# Autodesk Inventor assembly: ASY дренаж угольные
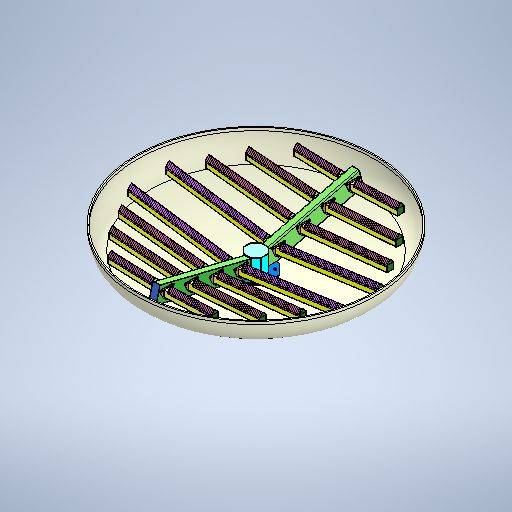
[picture p0: Inventor's stored thumbnail of the model, 512x512]
Saved by Autodesk Inventor 2025.1 (Build 291241020, 241B)
## iProperties
Created: 2024-12-09
Part Number: ASY дренаж угольные
Document SubType Name: Assembly
Designer: user
Author: user
## Documents named in this file (15)
- C:\Users\user\YandexDisk-badmisterfox\home pc\Inventor\filter-distribution-system\ASY BOTTOM filter distribution system.iam
- C:\Users\user\YandexDisk-badmisterfox\home pc\Inventor\filter-distribution-system\drain flange.ipt
- C:\Users\user\YandexDisk-badmisterfox\home pc\Inventor\filter-distribution-system\dished head.ipt
- C:\Users\user\YandexDisk-badmisterfox\home pc\Inventor\filter-distribution-system\DS-B-102 ridge bottom.ipt
- C:\Users\user\YandexDisk-badmisterfox\home pc\Inventor\filter-distribution-system\DS-B-101 Axis.ipt
- C:\Users\user\YandexDisk-badmisterfox\home pc\Inventor\filter-distribution-system\DS-B-104 ridge end cap.ipt
- C:\Users\user\YandexDisk-badmisterfox\home pc\Inventor\filter-distribution-system\DS-B-103 Ridge top.ipt
- C:\Users\user\YandexDisk-badmisterfox\home pc\Inventor\filter-distribution-system\ASY DS-B beam 1.iam
- C:\Users\user\YandexDisk-badmisterfox\home pc\Inventor\filter-distribution-system\000 DS-B dimentions.ipt
- C:\Users\user\YandexDisk-badmisterfox\home pc\Inventor\filter-distribution-system\111 DS-B outer tube.ipt
- C:\Users\user\YandexDisk-badmisterfox\home pc\Inventor\filter-distribution-system\110 DS-B drain sustem flange.ipt
- C:\Users\user\YandexDisk-badmisterfox\home pc\Inventor\filter-distribution-system\ASY DS-B beam 2.iam
- C:\Users\user\YandexDisk-badmisterfox\home pc\Inventor\filter-distribution-system\ASY DS-B beam 3.iam
- C:\Users\user\YandexDisk-badmisterfox\home pc\Inventor\filter-distribution-system\ASY DS-B beam 4.iam
- C:\Users\user\YandexDisk-badmisterfox\home pc\Inventor\filter-distribution-system\210 DS-B Axis cap.ipt
## Components (30 placed, 16 different names)
1. 000 DS-B dimentions.ipt:1
2. dished head.ipt:1 — Mate:4, Flush:3, Flush:4, Rigid:36
3. MNT-CDF-501 box.ipt:1 — Mate:5, Flush:5, Mate:6, Rigid:42, Rigid:43, Rigid:44, Rigid:45, Rigid:46
4. drain flange.ipt:1 — Rigid:37
5. MNT-CDF-503  main tube 1.ipt:1 — Rigid:39, Mate:7, Rigid:50
6. MNT-CDF-503  main tube 1.ipt:2 — Mate:5, Rigid:38
7. MNT-CDF-501 box.ipt:2 — Mate:7, Mate:8, Mate:9, Rigid:47, Rigid:52, Rigid:57, Rigid:58, Rigid:59
8. MNT-CDF-602 CAP.ipt:1 — Rigid:49
9. MNT-CDF-602 CAP.ipt:2 — Rigid:48
10. MNT-CDF-603 CAP.ipt:2 — Rigid:46, Rigid:49, Rigid:54, Rigid:55, Rigid:56, Rigid:63
11. ASY CDF 1100 beam 1.iam:1 [sub-assembly] — Rigid:42
12. 000 DS-B outer tube.ipt:1 — Rigid:36, Rigid:37
13. 110 DS-B drain sustem flange.ipt:1 — Mate:6, Rigid:38, Rigid:39, Mate:8
14. ASY DS-B beam 2:1 [sub-assembly] — Rigid:43
15. ASY DS-B beam 3:1 [sub-assembly] — Rigid:44
16. ASY DS-B beam 4:1 [sub-assembly] — Rigid:45
17. MNT-CDF-603 CAP:3 — Rigid:47, Rigid:48, Rigid:53, Rigid:60, Rigid:61, Rigid:62
18. 210 DS-B Axis cap:1 — Rigid:50
19. ASY DS-B beam 1:2 [sub-assembly] — Rigid:63
20. ASY DS-B beam 1:3 [sub-assembly] — Rigid:52
21. ASY DS-B beam 1:4 [sub-assembly] — Rigid:53
22. ASY DS-B beam 2:2 [sub-assembly] — Rigid:54
23. ASY DS-B beam 3:2 [sub-assembly] — Rigid:55
24. ASY DS-B beam 4:2 [sub-assembly] — Rigid:56
25. ASY DS-B beam 2:3 [sub-assembly] — Rigid:57
26. ASY DS-B beam 3:3 [sub-assembly] — Rigid:58
27. ASY DS-B beam 4:3 [sub-assembly] — Rigid:59
28. ASY DS-B beam 2:4 [sub-assembly] — Rigid:60
29. ASY DS-B beam 3:4 [sub-assembly] — Rigid:61
30. ASY DS-B beam 4:4 [sub-assembly] — Rigid:62
## Relationships (34: WeldJoint 25, Mate 6, Flush 3)
- Mate:4: dished head.ipt:1
- Flush:3: dished head.ipt:1
- Flush:4: dished head.ipt:1
- Rigid:36 [WeldJoint]: dished head.ipt:1 ↔ 000 DS-B outer tube.ipt:1
- Rigid:37 [WeldJoint]: drain flange.ipt:1 ↔ 000 DS-B outer tube.ipt:1
- Mate:5: MNT-CDF-501 box.ipt:1 ↔ MNT-CDF-503  main tube 1.ipt:2
- Flush:5: MNT-CDF-501 box.ipt:1
- Mate:6: MNT-CDF-501 box.ipt:1 ↔ 110 DS-B drain sustem flange.ipt:1
- Rigid:38 [WeldJoint]: MNT-CDF-503  main tube 1.ipt:2 ↔ 110 DS-B drain sustem flange.ipt:1
- Rigid:39 [WeldJoint]: MNT-CDF-503  main tube 1.ipt:1 ↔ 110 DS-B drain sustem flange.ipt:1
- Mate:7: MNT-CDF-503  main tube 1.ipt:1 ↔ MNT-CDF-501 box.ipt:2
- Mate:8: MNT-CDF-501 box.ipt:2 ↔ 110 DS-B drain sustem flange.ipt:1
- Mate:9: MNT-CDF-501 box.ipt:2
- Rigid:42 [WeldJoint]: MNT-CDF-501 box.ipt:1 ↔ ASY CDF 1100 beam 1.iam:1
- Rigid:43 [WeldJoint]: MNT-CDF-501 box.ipt:1 ↔ ASY DS-B beam 2:1
- Rigid:44 [WeldJoint]: MNT-CDF-501 box.ipt:1 ↔ ASY DS-B beam 3:1
- Rigid:45 [WeldJoint]: MNT-CDF-501 box.ipt:1 ↔ ASY DS-B beam 4:1
- Rigid:46 [WeldJoint]: MNT-CDF-501 box.ipt:1 ↔ MNT-CDF-603 CAP.ipt:2
- Rigid:47 [WeldJoint]: MNT-CDF-501 box.ipt:2 ↔ MNT-CDF-603 CAP:3
- Rigid:48 [WeldJoint]: MNT-CDF-602 CAP.ipt:2 ↔ MNT-CDF-603 CAP:3
- Rigid:49 [WeldJoint]: MNT-CDF-602 CAP.ipt:1 ↔ MNT-CDF-603 CAP.ipt:2
- Rigid:50 [WeldJoint]: MNT-CDF-503  main tube 1.ipt:1 ↔ 210 DS-B Axis cap:1
- Rigid:52 [WeldJoint]: MNT-CDF-501 box.ipt:2 ↔ ASY DS-B beam 1:3
- Rigid:53 [WeldJoint]: MNT-CDF-603 CAP:3 ↔ ASY DS-B beam 1:4
- Rigid:54 [WeldJoint]: MNT-CDF-603 CAP.ipt:2 ↔ ASY DS-B beam 2:2
- Rigid:55 [WeldJoint]: MNT-CDF-603 CAP.ipt:2 ↔ ASY DS-B beam 3:2
- Rigid:56 [WeldJoint]: MNT-CDF-603 CAP.ipt:2 ↔ ASY DS-B beam 4:2
- Rigid:57 [WeldJoint]: MNT-CDF-501 box.ipt:2 ↔ ASY DS-B beam 2:3
- Rigid:58 [WeldJoint]: MNT-CDF-501 box.ipt:2 ↔ ASY DS-B beam 3:3
- Rigid:59 [WeldJoint]: MNT-CDF-501 box.ipt:2 ↔ ASY DS-B beam 4:3
- Rigid:60 [WeldJoint]: MNT-CDF-603 CAP:3 ↔ ASY DS-B beam 2:4
- Rigid:61 [WeldJoint]: MNT-CDF-603 CAP:3 ↔ ASY DS-B beam 3:4
- Rigid:62 [WeldJoint]: MNT-CDF-603 CAP:3 ↔ ASY DS-B beam 4:4
- Rigid:63 [WeldJoint]: MNT-CDF-603 CAP.ipt:2 ↔ ASY DS-B beam 1:2
